# Autodesk Inventor assembly: U-ROV_Assembly_WorkingDrawing
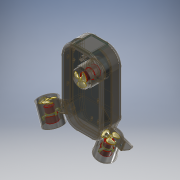
[picture p0: Inventor's stored thumbnail of the model, 180x180]
Saved by Autodesk Inventor 2019 (Build 230136000, 136)
## iProperties
Created: 2019-03-02
Part Number: U-ROV_Assembly_WorkingDrawing
Document SubType Name: Assembly
Designer: User
Author: User
## Documents named in this file (10)
- W:\CHAR NOTES\PROJECT\WORKING DRAWINGS\U-ROV_Assembly_WorkingDrawing.iam
- W:\CHAR NOTES\PROJECT\WORKING DRAWINGS\ROV Hull_Bottom Half 3.0.ipt
- W:\CHAR NOTES\PROJECT\WORKING DRAWINGS\ThrusterAssembly.iam
- C:\Users\User\Documents\Inventor\Content Center Files\R2019\en-US\SS-ISO 1207\ISO 1207 - M5 x 6SS-ISO.ipt
- C:\Users\User\Documents\Inventor\Content Center Files\R2019\en-US\BS EN 24 036\BS EN 24 036 - M3.5 _.ipt
- C:\Users\User\Documents\Inventor\Content Center Files\R2019\en-US\DIN 923\DIN 923 - M3 x 10.ipt
- W:\CHAR NOTES\PROJECT\WORKING DRAWINGS\Rear Thruster 2.0.ipt
- W:\CHAR NOTES\PROJECT\WORKING DRAWINGS\ROV Hull_Top Half 3.0.ipt
- W:\CHAR NOTES\PROJECT\WORKING DRAWINGS\Bilge-pump-motor.ipt
- W:\CHAR NOTES\PROJECT\WORKING DRAWINGS\Sight Glass.ipt
## Components (13 placed, 9 different names)
1. ROV Hull_Bottom Half 3.0:1 — Insert:1, Insert:2, Insert:3, Insert:4, Insert:5, Insert:6, Insert:7, Insert:8, Insert:9, Mate:1
2. ThrusterAssembly:1 [sub-assembly] — Insert:1
3. SS ISO 1207 M5 x 6:1 — Insert:2
4. SS ISO 1207 M5 x 6:2 — Insert:3
5. SS ISO 1207 M5 x 6:3 — Insert:4
6. SS ISO 1207 M5 x 6:4 — Insert:5
7. ThrusterAssembly:2 [sub-assembly] — Insert:6
8. Bilge-pump-motor:1 — Insert:7, Insert:10
9. DIN 923 M3 x 10:1 — Insert:8
10. BS EN 24036 M3.5 *:1 — Insert:9
11. Rear Thruster 2.0:1 — Insert:10
12. ROV Hull_Top Half 3.0:1 — Mate:1, Mate:2, Mate:3
13. Sight Glass:1 — Mate:2, Mate:3
## Relationships (13: Insert 10, Mate 3)
- Insert:1: ROV Hull_Bottom Half 3.0:1 ↔ ThrusterAssembly:1
- Insert:2: ROV Hull_Bottom Half 3.0:1 ↔ SS ISO 1207 M5 x 6:1
- Insert:3: ROV Hull_Bottom Half 3.0:1 ↔ SS ISO 1207 M5 x 6:2
- Insert:4: ROV Hull_Bottom Half 3.0:1 ↔ SS ISO 1207 M5 x 6:3
- Insert:5: ROV Hull_Bottom Half 3.0:1 ↔ SS ISO 1207 M5 x 6:4
- Insert:6: ROV Hull_Bottom Half 3.0:1 ↔ ThrusterAssembly:2
- Insert:7 (-28 mm): ROV Hull_Bottom Half 3.0:1 ↔ Bilge-pump-motor:1
- Insert:8: ROV Hull_Bottom Half 3.0:1 ↔ DIN 923 M3 x 10:1
- Insert:9: ROV Hull_Bottom Half 3.0:1 ↔ BS EN 24036 M3.5 *:1
- Insert:10 (-6 mm): Bilge-pump-motor:1 ↔ Rear Thruster 2.0:1
- Mate:1: ROV Hull_Bottom Half 3.0:1 ↔ ROV Hull_Top Half 3.0:1
- Mate:2: ROV Hull_Top Half 3.0:1 ↔ Sight Glass:1
- Mate:3: ROV Hull_Top Half 3.0:1 ↔ Sight Glass:1
